# Autodesk Inventor assembly: servo
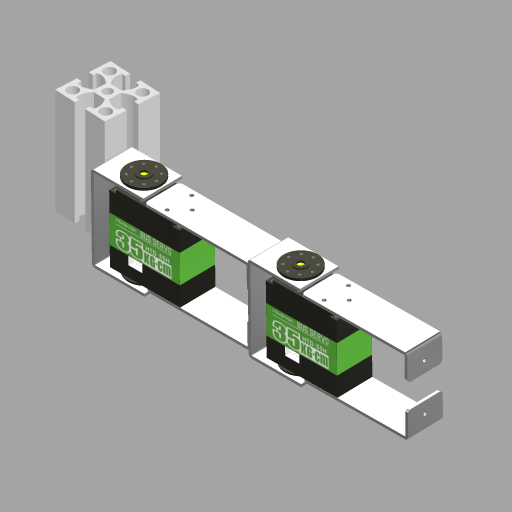
[picture p0: Inventor's stored thumbnail of the model, 512x512]
Saved by Autodesk Inventor 2023.1 (Build 271208000, 208)
## iProperties
Created: 2022-10-15
Part Number: servo
Document SubType Name: Assembly
Designer: 박동준
Author: 박동준
## Documents named in this file (8)
- C:\Users\박동준\OneDrive - 연세대학교 (Yonsei University)\바탕 화면\박동준\대학생할\로봇\Humanoid\Inventor_shared\2-Axis Manipulator\Designs\Assembly\servo.iam
- C:\Users\박동준\OneDrive - 연세대학교 (Yonsei University)\바탕 화면\박동준\대학생할\로봇\Humanoid\Inventor_shared\2-Axis Manipulator\Designs\Part\servo.ipt
- C:\Users\박동준\OneDrive - 연세대학교 (Yonsei University)\바탕 화면\박동준\대학생할\로봇\Humanoid\Inventor_shared\2-Axis Manipulator\Designs\Part\servo_bracket_bottom.ipt
- C:\Users\박동준\OneDrive - 연세대학교 (Yonsei University)\바탕 화면\박동준\대학생할\로봇\Humanoid\Inventor_shared\2-Axis Manipulator\Designs\Part\servo_bracket_top.ipt
- C:\Users\박동준\OneDrive - 연세대학교 (Yonsei University)\바탕 화면\박동준\대학생할\로봇\Humanoid\Inventor_shared\2-Axis Manipulator\Designs\Part\servo-horn_bottom.ipt
- C:\Users\박동준\OneDrive - 연세대학교 (Yonsei University)\바탕 화면\박동준\대학생할\로봇\Humanoid\Inventor_shared\2-Axis Manipulator\Designs\Part\servo-horn_top.ipt
- C:\Users\박동준\OneDrive - 연세대학교 (Yonsei University)\바탕 화면\박동준\대학생할\로봇\Humanoid\Inventor_shared\2-Axis Manipulator\Designs\Part\servo_horn_bracket.ipt
- C:\Users\박동준\OneDrive - 연세대학교 (Yonsei University)\바탕 화면\박동준\대학생할\로봇\Humanoid\Inventor_shared\2-Axis Manipulator\Designs\Part\3030 Aluminium Profile.ipt
## Components (13 placed, 7 different names)
1. servo:1 — 메이트:1, 메이트:2, 메이트:3, 메이트:4, 메이트:5, 메이트:8, 메이트:9, 메이트:10, 각도:1
2. servo_bracket_bottom:1 — 메이트:1, 메이트:4, 플러쉬:1, 각도:2, 각도:7
3. servo_bracket_top:1 — 메이트:2, 메이트:3, 플러쉬:1, 각도:3, 메이트:21, 메이트:22
4. servo-horn_bottom:1 — 메이트:8, 메이트:9, 각도:4
5. servo-horn_top:1 — 메이트:5, 메이트:10, 플러쉬:2, 메이트:23
6. servo_horn_bracket:1 — 플러쉬:2, 각도:5, 메이트:23
7. servo:2
8. servo_bracket_bottom:2
9. servo_bracket_top:2
10. servo-horn_bottom:2
11. servo-horn_top:2
12. servo_horn_bracket:2 — 메이트:21, 메이트:22, 각도:7
13. 3030 Aluminium Profile:1 — 각도:6
## Relationships (31: Mate 20, Angle 7, Flush 4)
- 메이트:1 [Mate] (0.05 mm): servo:1 ↔ servo_bracket_bottom:1
- 메이트:2 [Mate] (0.05 mm): servo:1 ↔ servo_bracket_top:1
- 메이트:3 [Mate]: servo:1 ↔ servo_bracket_top:1
- 메이트:4 [Mate]: servo:1 ↔ servo_bracket_bottom:1
- 메이트:5 [Mate]: servo:1 ↔ servo-horn_top:1
- 메이트:8 [Mate] (0.05 mm): servo:1 ↔ servo-horn_bottom:1
- 메이트:9 [Mate]: servo:1 ↔ servo-horn_bottom:1
- 메이트:10 [Mate] (0.05 mm): servo:1 ↔ servo-horn_top:1
- 플러쉬:1 [Flush]: servo_bracket_bottom:1 ↔ servo_bracket_top:1
- 플러쉬:2 [Flush] (1.3 mm): servo-horn_top:1 ↔ servo_horn_bracket:1
- [Mate] (0.05 mm): servo:2 ↔ servo_bracket_bottom:2
- [Mate] (0.05 mm): servo:2 ↔ servo_bracket_top:2
- [Mate]: servo:2 ↔ servo_bracket_top:2
- [Mate]: servo:2 ↔ servo_bracket_bottom:2
- [Mate]: servo:2 ↔ servo-horn_top:2
- [Mate] (0.05 mm): servo:2 ↔ servo-horn_bottom:2
- [Mate]: servo:2 ↔ servo-horn_bottom:2
- [Mate] (0.05 mm): servo:2 ↔ servo-horn_top:2
- [Flush]: servo_bracket_bottom:2 ↔ servo_bracket_top:2
- [Mate]: servo-horn_top:2 ↔ servo_horn_bracket:2
- [Flush] (1.3 mm): servo-horn_top:2 ↔ servo_horn_bracket:2
- 각도:1 [Angle] (0 deg): servo:1
- 각도:2 [Angle] (0 deg): servo_bracket_bottom:1
- 각도:3 [Angle] (0 deg): servo_bracket_top:1
- 각도:4 [Angle] (0 deg): servo-horn_bottom:1
- 각도:5 [Angle] (270 deg): servo_horn_bracket:1
- 각도:6 [Angle] (0 deg): 3030 Aluminium Profile:1
- 메이트:21 [Mate]: servo_bracket_top:1 ↔ servo_horn_bracket:2
- 메이트:22 [Mate]: servo_bracket_top:1 ↔ servo_horn_bracket:2
- 각도:7 [Angle] (0 deg): servo_bracket_bottom:1 ↔ servo_horn_bracket:2
- 메이트:23 [Mate]: servo-horn_top:1 ↔ servo_horn_bracket:1
## Named parameters: d27_d0 = 0.05 mm, d28_d1 = 0.05 mm, d29_d2 = 0 mm, d30_d3 = 0 mm, d31_d4 = 0 mm, d32_d7 = 0.05 mm, d33_d8 = 0 mm, d34_d9 = 0.05 mm, d35_d22 = 0 mm, d36_d24 = 1.3 mm, d37_d16 = 0 mm
